# Autodesk Inventor assembly: Femm
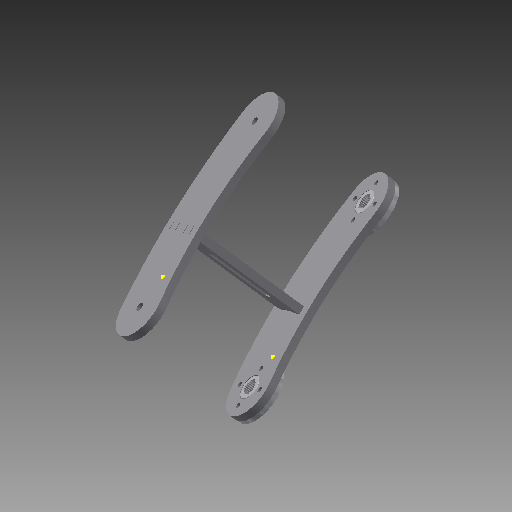
[picture p0: Inventor's stored thumbnail of the model, 512x512]
Saved by Autodesk Inventor 2019 (Build 230136000, 136)
## iProperties
Created: 2023-04-16
Part Number: Femm
Document SubType Name: Assembly
Designer: Analuam
Author: Analuam
## Documents named in this file (5)
- D:\Dek Diyah\Femm.iam
- D:\Dek Diyah\fem.ipt
- D:\Dek Diyah\fem2.ipt
- D:\Dek Diyah\HubFem.ipt
- D:\Dek Diyah\servomg996r\Acople circular.ipt
## Components (5 placed, 4 different names)
1. fem:1 — Insert:1, Mate:1, Mate:2, Mate:5, Insert:2
2. fem2:1 — Mate:3, Mate:4, Mate:6
3. HubFem:1 — Mate:1, Mate:2, Mate:3, Mate:4, Mate:5, Mate:6
4. Acople circular:1 — Insert:1
5. Acople circular:2 — Insert:2
## Relationships (8: Mate 6, Insert 2)
- Insert:1: fem:1 ↔ Acople circular:1
- Mate:1: fem:1 ↔ HubFem:1
- Mate:2: fem:1 ↔ HubFem:1
- Mate:3: fem2:1 ↔ HubFem:1
- Mate:4: fem2:1 ↔ HubFem:1
- Mate:5: fem:1 ↔ HubFem:1
- Mate:6: fem2:1 ↔ HubFem:1
- Insert:2: fem:1 ↔ Acople circular:2
